# Autodesk Inventor assembly: gyroGearHeadAssembly01
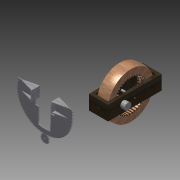
[picture p0: Inventor's stored thumbnail of the model, 180x180]
Saved by Autodesk Inventor 2013 (Build 170138000, 138)
## iProperties
Created: 2013-02-23
Part Number: gyroGearHeadAssembly01
Document SubType Name: Assembly
Designer: Nano
Author: Nano
## Documents named in this file (4)
- C:\Users\Nano\Documents\InventorByron\InventorMasterProject\gyroPhone01\gyroGearHeadAssembly01.iam
- C:\Users\Nano\Documents\InventorByron\InventorMasterProject\gyroPhone01\gear180_03.iam
- C:\Users\Nano\Documents\InventorByron\InventorMasterProject\gyroPhone01\motorWheelAssembly01.iam
- C:\Users\Nano\Documents\InventorByron\InventorMasterProject\gyroPhone01\gyroWheelCradle01.ipt
## Components (3 placed, 3 different names)
1. gear180_03:1 [sub-assembly]
2. motorWheelAssembly01:1 [sub-assembly] — Flush:1, Mate:1, Mate:2, Mate:3, Mate:4, Mate:5
3. gyroWheelCradle01:1 — Flush:1, Mate:1, Mate:2, Mate:3, Mate:4, Mate:5
## Relationships (6: Mate 5, Flush 1)
- Flush:1: motorWheelAssembly01:1 ↔ gyroWheelCradle01:1
- Mate:1: motorWheelAssembly01:1 ↔ gyroWheelCradle01:1
- Mate:2 (4.7625 mm): motorWheelAssembly01:1 ↔ gyroWheelCradle01:1
- Mate:3: motorWheelAssembly01:1 ↔ gyroWheelCradle01:1
- Mate:4 (4.7625 mm): motorWheelAssembly01:1 ↔ gyroWheelCradle01:1
- Mate:5 (5.842 mm): motorWheelAssembly01:1 ↔ gyroWheelCradle01:1
